# Autodesk Inventor assembly: PopulatedPCB
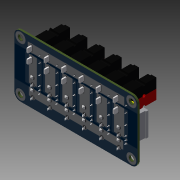
[picture p0: Inventor's stored thumbnail of the model, 180x180]
Saved by Autodesk Inventor 2014 SP1 (Build 180222100, 222)
## iProperties
Created: 2016-03-18
Part Number: PopulatedPCB
Document SubType Name: Assembly
Designer: Tyler
Author: Tyler
## Documents named in this file (8)
- C:\Users\Tyler\Documents\powerpolebreakout\Cad\PopulatedPCB.iam
- C:\Users\Tyler\Documents\powerpolebreakout\Cad\PCB.ipt
- C:\Users\Tyler\Documents\powerpolebreakout\Cad\PowerpolePairWContacts.iam
- C:\Users\Tyler\Documents\powerpolebreakout\Cad\FuseHolder.ipt
- C:\Users\Tyler\Documents\powerpolebreakout\Cad\ATCFuse.ipt
- C:\Users\Tyler\Documents\powerpolebreakout\Cad\LED3mm.ipt
- C:\Users\Tyler\Documents\powerpolebreakout\Cad\Resistor.ipt
- C:\Users\Tyler\Documents\powerpolebreakout\Cad\Capacitor.ipt
## Components (43 placed, 7 different names)
1. PCB:1 — Mate:1, Mate:12, Mate:13, Mate:16, Mate:17, Mate:18, Mate:20, Mate:21
2. PowerpolePairWContacts:1 [sub-assembly] — Mate:1, Flush:11, Mate:21
3. FuseHolder:1 — Mate:13, Flush:9, Flush:10
4. FuseHolder:2 — Mate:12, Flush:9, Flush:10, Mate:14, Mate:15
5. ATCFuse:1 — Mate:14, Mate:15, Mate:16, Flush:11, Mate:20
6. LED3mm:1 — Mate:18, Flush:12, Mate:19
7. Resistor:1 — Flush:12, Mate:19, Flush:13
8. Capacitor:1 — Flush:13
9. PowerpolePairWContacts:2 [sub-assembly]
10. FuseHolder:3
11. FuseHolder:4
12. ATCFuse:2
13. LED3mm:2
14. Resistor:2
15. Capacitor:2
16. PowerpolePairWContacts:3 [sub-assembly] — Mate:17
17. FuseHolder:5
18. FuseHolder:6
19. ATCFuse:3
20. LED3mm:3
21. Resistor:3
22. Capacitor:3
23. PowerpolePairWContacts:4 [sub-assembly]
24. FuseHolder:7
25. FuseHolder:8
26. ATCFuse:4
27. LED3mm:4
28. Resistor:4
29. Capacitor:4
30. PowerpolePairWContacts:5 [sub-assembly]
31. FuseHolder:9
32. FuseHolder:10
33. ATCFuse:5
34. LED3mm:5
35. Resistor:5
36. Capacitor:5
37. PowerpolePairWContacts:6 [sub-assembly]
38. FuseHolder:11
39. FuseHolder:12
40. ATCFuse:6
41. LED3mm:6
42. Resistor:6
43. Capacitor:6
## Component patterns: (6 elements, first: PowerpolePairWContacts:1 + FuseHolder:1 + FuseHolder:2 + ATCFuse:1 + LED3mm:1 + Resistor:1 + Capacitor:1)
## Relationships (16: Mate 11, Flush 5)
- Mate:1: PCB:1 ↔ PowerpolePairWContacts:1
- Mate:12: PCB:1 ↔ FuseHolder:2
- Mate:13: PCB:1 ↔ FuseHolder:1
- Flush:9: FuseHolder:1 ↔ FuseHolder:2
- Flush:10 (9.2 mm): FuseHolder:1 ↔ FuseHolder:2
- Mate:14 (-4.6 mm): FuseHolder:2 ↔ ATCFuse:1
- Mate:15: FuseHolder:2 ↔ ATCFuse:1
- Mate:16 (1 mm): PCB:1 ↔ ATCFuse:1
- Flush:11 (0.5 mm): PowerpolePairWContacts:1 ↔ ATCFuse:1
- Mate:17 (-7 mm): PCB:1 ↔ PowerpolePairWContacts:3
- Mate:18: PCB:1 ↔ LED3mm:1
- Flush:12: LED3mm:1 ↔ Resistor:1
- Mate:19: LED3mm:1 ↔ Resistor:1
- Flush:13: Resistor:1 ↔ Capacitor:1
- Mate:20 (-15 mm): PCB:1 ↔ ATCFuse:1
- Mate:21 (-12 mm): PCB:1 ↔ PowerpolePairWContacts:1
